# Autodesk Inventor assembly: Assembly_water
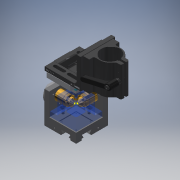
[picture p0: Inventor's stored thumbnail of the model, 180x180]
Saved by Autodesk Inventor 2018 (Build 220112000, 112)
## iProperties
Created: 2018-08-29
Part Number: Assembly_water
Document SubType Name: Assembly
Designer: David
Author: David
## Documents named in this file (11)
- C:\Users\David\Documents\optoelectronics\LightSheetMicroscope\Printing\Assembly_water.iam
- C:\Users\David\Documents\optoelectronics\LightSheetMicroscope\Printing\sample_holder.ipt
- C:\Users\David\Documents\optoelectronics\LightSheetMicroscope\Printing\objective.ipt
- C:\Users\David\Documents\optoelectronics\LightSheetMicroscope\Printing\brain_holder.ipt
- C:\Users\David\Documents\optoelectronics\LightSheetMicroscope\Printing\modified_o_ring.ipt
- C:\Users\David\Documents\optoelectronics\LightSheetMicroscope\Printing\tester.ipt
- C:\Users\David\Documents\optoelectronics\LightSheetMicroscope\Printing\chamber.ipt
- C:\Users\David\Documents\optoelectronics\LightSheetMicroscope\tube holder\C1515_M-Step.ipt
- C:\Users\David\Documents\optoelectronics\LightSheetMicroscope\tube holder\motor upper holder.ipt
- C:\Users\David\Documents\optoelectronics\LightSheetMicroscope\tube holder\syringe holder.ipt
- C:\Users\David\Documents\optoelectronics\LightSheetMicroscope\Printing\actuator.ipt
## Components (11 placed, 10 different names)
1. sample_holder:1 — Mate:4, Mate:5, Flush:2, Flush:3, Mate:15, Mate:16, Mate:17, Mate:18, Flush:4, Flush:5, Mate:19, Mate:20, Mate:21
2. objective:1 — Mate:4, Flush:3, Mate:13
3. objective:2 — Mate:5, Flush:2, Mate:14
4. brain_holder:1 — Mate:13, Mate:14
5. modified_o_ring:1 — Mate:15, Mate:16, Mate:17
6. tester:1 — Mate:18, Flush:4, Flush:5
7. chamber:1 — Mate:19, Mate:20, Mate:21, Mate:22
8. C1515_M-Step:1 — Mate:26, Mate:27, Mate:28
9. motor upper holder:1 — Mate:24, Mate:25, Mate:26, Mate:27, Mate:28
10. syringe holder:1 — Mate:22, Mate:23, Flush:6, Flush:7
11. actuator:1 — Mate:23, Flush:6, Flush:7, Mate:24, Mate:25
## Relationships (24: Mate 18, Flush 6)
- Mate:4: sample_holder:1 ↔ objective:1
- Mate:5: sample_holder:1 ↔ objective:2
- Flush:2: sample_holder:1 ↔ objective:2
- Flush:3: sample_holder:1 ↔ objective:1
- Mate:13 (5 mm): objective:1 ↔ brain_holder:1
- Mate:14 (5 mm): objective:2 ↔ brain_holder:1
- Mate:15: sample_holder:1 ↔ modified_o_ring:1
- Mate:16: sample_holder:1 ↔ modified_o_ring:1
- Mate:17: sample_holder:1 ↔ modified_o_ring:1
- Mate:18: sample_holder:1 ↔ tester:1
- Flush:4: sample_holder:1 ↔ tester:1
- Flush:5 (9.5 mm): sample_holder:1 ↔ tester:1
- Mate:19: sample_holder:1 ↔ chamber:1
- Mate:20: sample_holder:1 ↔ chamber:1
- Mate:21: sample_holder:1 ↔ chamber:1
- Mate:22 (20 mm): chamber:1 ↔ syringe holder:1
- Mate:23: syringe holder:1 ↔ actuator:1
- Flush:6: syringe holder:1 ↔ actuator:1
- Flush:7: syringe holder:1 ↔ actuator:1
- Mate:24: motor upper holder:1 ↔ actuator:1
- Mate:25: motor upper holder:1 ↔ actuator:1
- Mate:26: C1515_M-Step:1 ↔ motor upper holder:1
- Mate:27: C1515_M-Step:1 ↔ motor upper holder:1
- Mate:28: C1515_M-Step:1 ↔ motor upper holder:1
